# Autodesk Inventor assembly: tolva completa
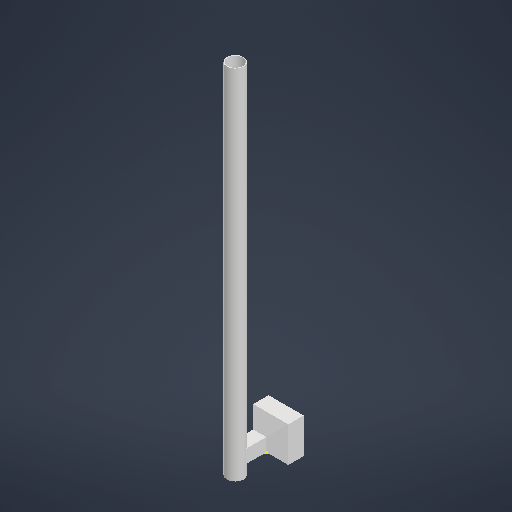
[picture p0: Inventor's stored thumbnail of the model, 512x512]
Saved by Autodesk Inventor 2026.1 (Build 301233020, 233B)
## iProperties
Created: 2025-12-03
Part Number: tolva completa
Document SubType Name: Assembly
Designer: benja
Author: benja
## Documents named in this file (3)
- C:\Users\benja\OneDrive\Escritorio\extrusora\tolva completa.iam
- C:\Users\benja\OneDrive\Escritorio\extrusora\tolva.ipt
- C:\Users\benja\OneDrive\Escritorio\extrusora\tubo cubierta tornillo.ipt
## Components (2 placed, 2 different names)
1. tolva:1 — Coincidencia:1, Coincidencia:2, Coincidencia:3, Coincidencia:4, Coincidencia:5
2. tubo cubierta tornillo:1 — Coincidencia:1, Coincidencia:2, Coincidencia:3, Coincidencia:4, Coincidencia:5
## Relationships (5: Mate 5)
- Coincidencia:1 [Mate]: tolva:1 ↔ tubo cubierta tornillo:1
- Coincidencia:2 [Mate]: tolva:1 ↔ tubo cubierta tornillo:1
- Coincidencia:3 [Mate]: tolva:1 ↔ tubo cubierta tornillo:1
- Coincidencia:4 [Mate]: tolva:1 ↔ tubo cubierta tornillo:1
- Coincidencia:5 [Mate]: tolva:1 ↔ tubo cubierta tornillo:1
